# Autodesk Inventor assembly: SecuroBot Assembly
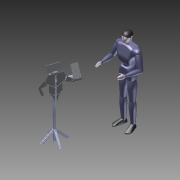
[picture p0: Inventor's stored thumbnail of the model, 180x180]
Saved by Autodesk Inventor 2014 SP2 (Build 180246200, 246)
## iProperties
Created: 2015-07-31
Part Number: SecuroBot Assembly
Document SubType Name: Assembly
Designer: Devon
Author: Devon
## Documents named in this file (24)
- C:\Users\Devon\Dropbox\Devon\Graduate\UNH CFREG\SecuroBot Assembly.iam
- C:\Users\Devon\Dropbox\Devon\Graduate\UNH CFREG\Big Leg.ipt
- C:\Users\Devon\Dropbox\Devon\Graduate\UNH CFREG\Spine.ipt
- C:\Users\Devon\Dropbox\Devon\Graduate\UNH CFREG\Left Arm.ipt
- C:\Users\Devon\Dropbox\Devon\Graduate\UNH CFREG\Rotating Base mount.ipt
- C:\Users\Devon\Dropbox\Devon\Graduate\UNH CFREG\Rotating Base.ipt
- C:\Users\Devon\Dropbox\Devon\Graduate\UNH CFREG\Imported Components\ANGLE BRACE\ANGLE BRACE.ipt
- C:\Users\Devon\Dropbox\Devon\Graduate\UNH CFREG\Imported Components\person\person.ipt
- C:\Users\Devon\Dropbox\Devon\Graduate\UNH CFREG\Imported Components\enclosure\enclosure.ipt
- C:\Users\Devon\Dropbox\Devon\Graduate\UNH CFREG\Left Abdomen.ipt
- C:\Users\Devon\Dropbox\Devon\Graduate\UNH CFREG\Left Chest.ipt
- C:\Users\Devon\Dropbox\Devon\Graduate\UNH CFREG\Left Hip.ipt
- C:\Users\Devon\Dropbox\Devon\Graduate\UNH CFREG\Right Abdomen.ipt
- C:\Users\Devon\Dropbox\Devon\Graduate\UNH CFREG\Right Chest.ipt
- C:\Users\Devon\Dropbox\Devon\Graduate\UNH CFREG\Right Hip.ipt
- C:\Users\Devon\Dropbox\Devon\Graduate\UNH CFREG\Left Bicep.ipt
- C:\Users\Devon\Dropbox\Devon\Graduate\UNH CFREG\Left Forearm.ipt
- C:\Users\Devon\Dropbox\Devon\Graduate\UNH CFREG\Right Bicep.ipt
- C:\Users\Devon\Dropbox\Devon\Graduate\UNH CFREG\Right Forearm.ipt
- C:\Users\Devon\Dropbox\Devon\Graduate\UNH CFREG\Master Tablet Cover.ipt
- C:\Users\Devon\Dropbox\Devon\Graduate\UNH CFREG\Master Tablet Enclosure.ipt
- C:\Users\Devon\Dropbox\Devon\Graduate\UNH CFREG\Slave Tablet Cover.ipt
- C:\Users\Devon\Dropbox\Devon\Graduate\UNH CFREG\Slave Tablet Enclosure.ipt
- C:\Users\Devon\Documents\Inventor\small angle brace.ipt
## Components (29 placed, 23 different names)
1. Big Leg:1 — Mate:2, Flush:3, Flush:4
2. Spine:1 — Mate:2, Flush:3, Flush:4, Mate:4, Flush:7, Flush:8, Mate:5, Flush:9, Flush:10, Mate:6, Flush:11, Flush:12, Mate:7, Flush:13, Mate:10, Flush:16, Mate:13, Flush:17, Mate:14, Flush:18, Mate:16, Flush:19, Insert:1, Mate:42, Mate:43, Mate:45, Mate:46, Flush:31, Flush:32, Mate:47, Flush:33, Mate:49, Flush:34, Mate:51, Mate:52, Flush:35, Flush:36, Mate:78, Flush:51
3. Big Leg:2 — Mate:4, Flush:7, Flush:8, Flush:27
4. Big Leg:3 — Mate:5, Flush:9, Flush:10
5. Big Leg:4 — Mate:6, Flush:11, Flush:12
6. Left Arm:1 — Mate:7, Flush:13, Mate:55, Flush:37, Mate:57, Flush:38, Mate:76, Mate:77
7. Rotating Base mount:1 — Mate:9, Flush:14, Flush:15, Mate:11, Mate:12, Mate:15, Mate:17, Insert:1
8. Rotating Base:1 — Mate:9, Flush:14, Flush:15, Flush:29, Flush:30, Mate:74
9. ANGLE BRACE:1 — Mate:14, Mate:15, Flush:18, Mate:44
10. ANGLE BRACE:2 — Mate:12, Mate:13, Flush:17
11. ANGLE BRACE:3 — Mate:10, Mate:11, Flush:16
12. ANGLE BRACE:4 — Mate:16, Mate:17, Flush:19
13. person:1 — Flush:27
14. enclosure:1 — Mate:42, Mate:43, Mate:44
15. Left Abdomen:1 — Mate:47, Flush:33, Mate:48, Mate:53
16. Left Chest:1 — Mate:45, Flush:29, Flush:31, Mate:48, Mate:56, Mate:66
17. Left Hip:1 — Mate:51, Flush:36, Mate:53
18. Right Abdomen:1 — Mate:49, Flush:34, Mate:50, Mate:54
19. Right Chest:1 — Mate:46, Flush:30, Flush:32, Mate:50, Mate:59, Mate:60, Flush:39
20. Right Hip:1 — Mate:52, Flush:35, Mate:54
21. Left Bicep:1 — Mate:55, Mate:56, Flush:37, Mate:58, Mate:66
22. Left Forearm:1 — Mate:57, Flush:38, Mate:58, Mate:75, Flush:50
23. Right Bicep:1 — Mate:59, Mate:60, Flush:39, Flush:40, Mate:61, Flush:41
24. Right Forearm:1 — Flush:40, Mate:61, Flush:41
25. Master Tablet Cover:1 — Mate:65, Flush:44, Flush:45
26. Master Tablet Enclosure:1 — Mate:65, Flush:44, Flush:45, Mate:74
27. Slave Tablet Cover:1 — Mate:71, Flush:48, Flush:49
28. Slave Tablet Enclosure:1 — Mate:71, Flush:48, Flush:49, Mate:75, Mate:76, Flush:50
29. small angle brace:1 — Mate:77, Mate:78, Flush:51
## Relationships (78: Mate 42, Flush 35, Insert 1)
- Mate:2: Big Leg:1 ↔ Spine:1
- Flush:3: Big Leg:1 ↔ Spine:1
- Flush:4: Big Leg:1 ↔ Spine:1
- Mate:4: Spine:1 ↔ Big Leg:2
- Flush:7: Spine:1 ↔ Big Leg:2
- Flush:8: Spine:1 ↔ Big Leg:2
- Mate:5: Spine:1 ↔ Big Leg:3
- Flush:9: Spine:1 ↔ Big Leg:3
- Flush:10: Spine:1 ↔ Big Leg:3
- Mate:6: Spine:1 ↔ Big Leg:4
- Flush:11: Spine:1 ↔ Big Leg:4
- Flush:12: Spine:1 ↔ Big Leg:4
- Mate:7: Spine:1 ↔ Left Arm:1
- Flush:13: Spine:1 ↔ Left Arm:1
- Mate:9: Rotating Base mount:1 ↔ Rotating Base:1
- Flush:14: Rotating Base mount:1 ↔ Rotating Base:1
- Flush:15: Rotating Base mount:1 ↔ Rotating Base:1
- Mate:10: Spine:1 ↔ ANGLE BRACE:3
- Mate:11: Rotating Base mount:1 ↔ ANGLE BRACE:3
- Flush:16: Spine:1 ↔ ANGLE BRACE:3
- Mate:12: Rotating Base mount:1 ↔ ANGLE BRACE:2
- Mate:13: Spine:1 ↔ ANGLE BRACE:2
- Flush:17: Spine:1 ↔ ANGLE BRACE:2
- Mate:14: Spine:1 ↔ ANGLE BRACE:1
- Mate:15: Rotating Base mount:1 ↔ ANGLE BRACE:1
- Flush:18: Spine:1 ↔ ANGLE BRACE:1
- Mate:16: Spine:1 ↔ ANGLE BRACE:4
- Mate:17: Rotating Base mount:1 ↔ ANGLE BRACE:4
- Flush:19: Spine:1 ↔ ANGLE BRACE:4
- Insert:1: Spine:1 ↔ Rotating Base mount:1
- Flush:27: Big Leg:2 ↔ person:1
- Mate:42: Spine:1 ↔ enclosure:1
- Mate:43 (31.75 mm): Spine:1 ↔ enclosure:1
- Mate:44 (76.2 mm): ANGLE BRACE:1 ↔ enclosure:1
- Mate:45: Spine:1 ↔ Left Chest:1
- Mate:46: Spine:1 ↔ Right Chest:1
- Flush:29: Rotating Base:1 ↔ Left Chest:1
- Flush:30: Rotating Base:1 ↔ Right Chest:1
- Flush:31: Spine:1 ↔ Left Chest:1
- Flush:32: Spine:1 ↔ Right Chest:1
- Mate:47: Spine:1 ↔ Left Abdomen:1
- Flush:33: Spine:1 ↔ Left Abdomen:1
- Mate:48 (12.7 mm): Left Abdomen:1 ↔ Left Chest:1
- Mate:49: Spine:1 ↔ Right Abdomen:1
- Flush:34: Spine:1 ↔ Right Abdomen:1
- Mate:50 (12.7 mm): Right Abdomen:1 ↔ Right Chest:1
- Mate:51: Spine:1 ↔ Left Hip:1
- Mate:52: Spine:1 ↔ Right Hip:1
- Flush:35: Spine:1 ↔ Right Hip:1
- Flush:36: Spine:1 ↔ Left Hip:1
- Mate:53 (12.7 mm): Left Abdomen:1 ↔ Left Hip:1
- Mate:54 (12.7 mm): Right Abdomen:1 ↔ Right Hip:1
- Mate:55: Left Arm:1 ↔ Left Bicep:1
- Mate:56 (12.7 mm): Left Chest:1 ↔ Left Bicep:1
- Flush:37: Left Arm:1 ↔ Left Bicep:1
- Mate:57: Left Arm:1 ↔ Left Forearm:1
- Flush:38: Left Arm:1 ↔ Left Forearm:1
- Mate:58 (12.7 mm): Left Bicep:1 ↔ Left Forearm:1
- Mate:59: Right Chest:1 ↔ Right Bicep:1
- Mate:60: Right Chest:1 ↔ Right Bicep:1
- Flush:39: Right Chest:1 ↔ Right Bicep:1
- Flush:40: Right Bicep:1 ↔ Right Forearm:1
- Mate:61: Right Bicep:1 ↔ Right Forearm:1
- Flush:41: Right Bicep:1 ↔ Right Forearm:1
- Mate:65: Master Tablet Cover:1 ↔ Master Tablet Enclosure:1
- Flush:44: Master Tablet Cover:1 ↔ Master Tablet Enclosure:1
- Flush:45: Master Tablet Cover:1 ↔ Master Tablet Enclosure:1
- Mate:66 (12.7 mm): Left Chest:1 ↔ Left Bicep:1
- Mate:71: Slave Tablet Cover:1 ↔ Slave Tablet Enclosure:1
- Flush:48: Slave Tablet Cover:1 ↔ Slave Tablet Enclosure:1
- Flush:49: Slave Tablet Cover:1 ↔ Slave Tablet Enclosure:1
- Mate:74: Rotating Base:1 ↔ Master Tablet Enclosure:1
- Mate:75: Left Forearm:1 ↔ Slave Tablet Enclosure:1
- Mate:76: Left Arm:1 ↔ Slave Tablet Enclosure:1
- Flush:50: Left Forearm:1 ↔ Slave Tablet Enclosure:1
- Mate:77: Left Arm:1 ↔ small angle brace:1
- Mate:78: Spine:1 ↔ small angle brace:1
- Flush:51: Spine:1 ↔ small angle brace:1
